# Autodesk Inventor assembly: PROTOTIPO 2
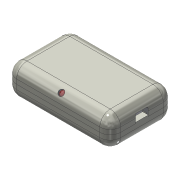
[picture p0: Inventor's stored thumbnail of the model, 180x180]
Saved by Autodesk Inventor 2022.1 (Build 261234020, 234B)
## iProperties
Created: 2022-10-28
Part Number: PROTOTIPO 2
Document SubType Name: Assembly
Designer: HP
Author: HP
## Documents named in this file (7)
- C:\Users\HP\OneDrive\Documentos\Inventor\BIODEÑO\Dispositivo 3-1.iam
- C:\Users\HP\OneDrive\Documentos\Inventor\BIODEÑO\CARCASA NUEVA.ipt
- C:\Users\HP\OneDrive\Documentos\Inventor\BIODEÑO\MINIPROTOBOARD.ipt
- C:\Users\HP\OneDrive\Documentos\Inventor\BIODEÑO\HX711.ipt
- C:\Users\HP\OneDrive\Documentos\Inventor\BIODEÑO\ESP-WROOM32.ipt
- C:\Users\HP\OneDrive\Documentos\Inventor\BIODEÑO\CARCASA NUEVA ARRIBA.ipt
- C:\Users\HP\OneDrive\Documentos\Inventor\BIODEÑO\LED 5mm.ipt
## Components (6 placed, 6 different names)
1. CARCASA NUEVA:1 — Mate:1, Mate:2, Mate:3, Flush:1, Flush:2, Mate:4
2. MINIPROTOBOARD:1 — Mate:1, Mate:2, Mate:3
3. HX711:1
4. ESP-WROOM32:1
5. CARCASA NUEVA ARRIBA:1 — Flush:1, Flush:2, Mate:4, Mate:5
6. LED 5mm:1 — Mate:5
## Relationships (7: Mate 5, Flush 2)
- Mate:1: CARCASA NUEVA:1 ↔ MINIPROTOBOARD:1
- Mate:2: CARCASA NUEVA:1 ↔ MINIPROTOBOARD:1
- Mate:3: CARCASA NUEVA:1 ↔ MINIPROTOBOARD:1
- Flush:1: CARCASA NUEVA:1 ↔ CARCASA NUEVA ARRIBA:1
- Flush:2: CARCASA NUEVA:1 ↔ CARCASA NUEVA ARRIBA:1
- Mate:4: CARCASA NUEVA:1 ↔ CARCASA NUEVA ARRIBA:1
- Mate:5: CARCASA NUEVA ARRIBA:1 ↔ LED 5mm:1
